# Autodesk Inventor assembly: Conjunto motor-polea
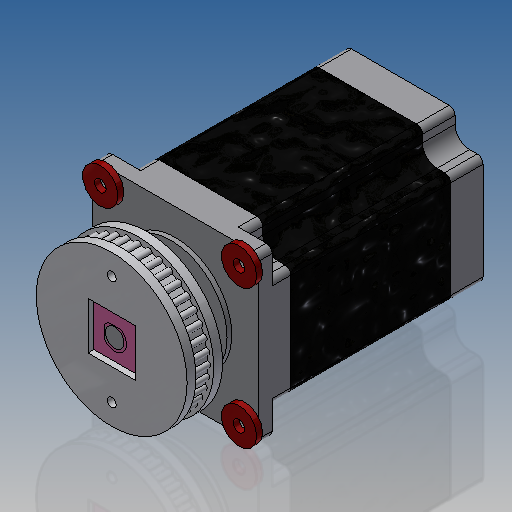
[picture p0: Inventor's stored thumbnail of the model, 512x512]
Saved by Autodesk Inventor 2017 (Build 210142000, 142)
## iProperties
Part Number: Conjunto motor-polea
Material: Genérico
Document SubType Name: Assembly
Designer: FABLAB
Author: FABLAB
## Documents named in this file (4)
- C:\Users\Leo\Documents\GitHub\actor-re-actor\models\inventor-caja\transmision Engranajes\Potencia.iam
- C:\Users\Leo\Documents\GitHub\actor-re-actor\models\inventor-caja\Piezas\Motor.ipt
- C:\Users\Leo\Documents\GitHub\actor-re-actor\models\inventor-caja\Piezas\golilla de goma.ipt
- C:\Users\Leo\Documents\GitHub\actor-re-actor\models\inventor-caja\transmision Engranajes\Polea motor.iam
## Components (6 placed, 3 different names)
1. Motor:1 — Insertar:1, Insertar:2, Insertar:3, Insertar:4, Insertar:5
2. Polea motor:1 [sub-assembly] — Insertar:1
3. golilla de goma:1 — Insertar:5
4. golilla de goma:2 — Insertar:4
5. golilla de goma:3 — Insertar:2
6. golilla de goma:4 — Insertar:3
## Relationships (5: Insert 5)
- Insertar:1: Motor:1 ↔ Polea motor:1
- Insertar:2: Motor:1 ↔ golilla de goma:3
- Insertar:3: Motor:1 ↔ golilla de goma:4
- Insertar:4: Motor:1 ↔ golilla de goma:2
- Insertar:5: Motor:1 ↔ golilla de goma:1
